# Autodesk Inventor assembly: Cartridge Full
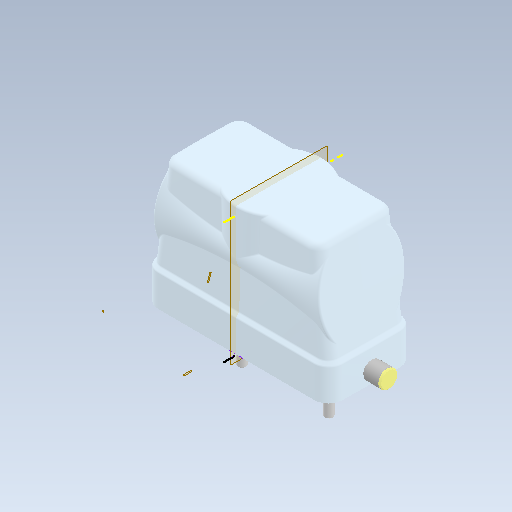
[picture p0: Inventor's stored thumbnail of the model, 512x512]
Saved by Autodesk Inventor 2021 (Build 250183000, 183)
## iProperties
Created: 2020-04-28
Part Number: Cartridge Full
Document SubType Name: Assembly
Designer: jgray
Author: jgray
## Documents named in this file (7)
- M:\Printed Electronics\Gas Sensors\Prototypes\Prototype II -Cartridge Reader V2\Cartridge Interface V5 30-06-20\Cartridge Full.iam
- M:\Printed Electronics\Gas Sensors\Prototypes\Prototype II -Cartridge Reader V2\Cartridge Interface V5 30-06-20\Cartridge Assembly 2.iam
- M:\Printed Electronics\Gas Sensors\Prototypes\Prototype II -Cartridge Reader V2\Cartridge Interface V5 30-06-20\Cartridge Enclosure1460102.iam
- M:\Printed Electronics\Gas Sensors\Prototypes\Prototype II -Cartridge Reader V2\Cartridge Interface V5 30-06-20\Cartridge Gland Seal M25 RS 664 4628.ipt
- M:\Printed Electronics\Gas Sensors\Prototypes\Prototype II -Cartridge Reader V2\Cartridge Interface V5 30-06-20\Cartridge Glans Cover RS 406-9413 LAPP.ipt
- M:\Printed Electronics\Gas Sensors\Prototypes\Prototype II -Cartridge Reader V2\Cartridge Interface V5 30-06-20\DIN 7985 (H) - M3x16-H.ipt
- M:\Printed Electronics\Gas Sensors\Prototypes\Prototype II -Cartridge Reader V2\Cartridge Interface V5 30-06-20\DIN 6798 - J 3.2.ipt
## Components (12 placed, 6 different names)
1. Cartridge Assembly 2:1 [sub-assembly] — Mate:1, Mate:2, Mate:3, Mate:23, Mate:24, Mate:25, Mate:26
2. Cartridge Enclosure1460102:1 [sub-assembly] — Mate:1, Mate:2, Mate:3, Mate:12, Mate:13, Mate:14, Mate:15, Mate:21, Mate:22
3. DIN 6798 J J 3.2:1 — Mate:5, Mate:9, Mate:24
4. DIN 6798 J J 3.2:2 — Mate:7, Mate:10, Mate:26
5. DIN 6798 J J 3.2:3 — Mate:4, Mate:8, Mate:23
6. DIN 6798 J J 3.2:4 — Mate:6, Mate:11, Mate:25
7. DIN 7985 (H) M3x16-H:1 — Mate:4, Mate:8, Mate:12
8. DIN 7985 (H) M3x16-H:2 — Mate:5, Mate:9, Mate:14
9. DIN 7985 (H) M3x16-H:3 — Mate:6, Mate:11, Mate:13
10. DIN 7985 (H) M3x16-H:4 — Mate:7, Mate:10, Mate:15
11. Cartridge Gland Seal M25 RS 664 4628:1 — Mate:20, Tangent:1
12. Cartridge Glans Cover RS 406-9413 LAPP:1 — Mate:20, Tangent:1, Mate:21, Mate:22
## Relationships (23: Mate 22, Tangent 1)
- Mate:1: Cartridge Assembly 2:1 ↔ Cartridge Enclosure1460102:1
- Mate:2: Cartridge Assembly 2:1 ↔ Cartridge Enclosure1460102:1
- Mate:3: Cartridge Assembly 2:1 ↔ Cartridge Enclosure1460102:1
- Mate:4: DIN 6798 J J 3.2:3 ↔ DIN 7985 (H) M3x16-H:1
- Mate:5: DIN 6798 J J 3.2:1 ↔ DIN 7985 (H) M3x16-H:2
- Mate:6: DIN 6798 J J 3.2:4 ↔ DIN 7985 (H) M3x16-H:3
- Mate:7: DIN 6798 J J 3.2:2 ↔ DIN 7985 (H) M3x16-H:4
- Mate:8: DIN 6798 J J 3.2:3 ↔ DIN 7985 (H) M3x16-H:1
- Mate:9: DIN 6798 J J 3.2:1 ↔ DIN 7985 (H) M3x16-H:2
- Mate:10: DIN 6798 J J 3.2:2 ↔ DIN 7985 (H) M3x16-H:4
- Mate:11: DIN 6798 J J 3.2:4 ↔ DIN 7985 (H) M3x16-H:3
- Mate:12: Cartridge Enclosure1460102:1 ↔ DIN 7985 (H) M3x16-H:1
- Mate:13: Cartridge Enclosure1460102:1 ↔ DIN 7985 (H) M3x16-H:3
- Mate:14: Cartridge Enclosure1460102:1 ↔ DIN 7985 (H) M3x16-H:2
- Mate:15: Cartridge Enclosure1460102:1 ↔ DIN 7985 (H) M3x16-H:4
- Mate:20: Cartridge Gland Seal M25 RS 664 4628:1 ↔ Cartridge Glans Cover RS 406-9413 LAPP:1
- Tangent:1: Cartridge Gland Seal M25 RS 664 4628:1 ↔ Cartridge Glans Cover RS 406-9413 LAPP:1
- Mate:21: Cartridge Enclosure1460102:1 ↔ Cartridge Glans Cover RS 406-9413 LAPP:1
- Mate:22 (1.4 mm): Cartridge Enclosure1460102:1 ↔ Cartridge Glans Cover RS 406-9413 LAPP:1
- Mate:23: Cartridge Assembly 2:1 ↔ DIN 6798 J J 3.2:3
- Mate:24: Cartridge Assembly 2:1 ↔ DIN 6798 J J 3.2:1
- Mate:25: Cartridge Assembly 2:1 ↔ DIN 6798 J J 3.2:4
- Mate:26: Cartridge Assembly 2:1 ↔ DIN 6798 J J 3.2:2
